# Autodesk Inventor assembly: Ensamblaje_eslabón
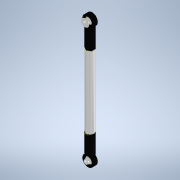
[picture p0: Inventor's stored thumbnail of the model, 180x180]
Saved by Autodesk Inventor 2020 (Build 240168000, 168)
## iProperties
Created: 2019-10-01
Part Number: Ensamblaje_eslabón
Document SubType Name: Assembly
Designer: Frederich Schnëider
Author: Frederich Schnëider
## Documents named in this file (5)
- C:\Users\Frederich Schnëider\Documents\Inventor\Eslabón TRA\Ensamblaje_eslabón.iam
- C:\Users\Frederich Schnëider\Documents\Inventor\Eslabón TRA\RCT-T003.ipt
- C:\Users\Frederich Schnëider\Documents\Inventor\Eslabón TRA\H016.ipt
- C:\Users\Frederich Schnëider\Documents\Inventor\Eslabón TRA\H016 (2).ipt
- C:\Users\Frederich Schnëider\Documents\Inventor\Eslabón TRA\RCT-T003 (2).ipt
## Components (5 placed, 4 different names)
1. RCT-T003:1 — De rotación:1, De rotación:2
2. RCT-T003 (2):1 — De rotación:2, De bola:1
3. RCT-T003 (2):2 — De rotación:1, De bola:2
4. H016:1 — De bola:2
5. H016 (2):1 — De bola:1
## Relationships (4: RevoluteJoint 2, BallJoint 2)
- De rotación:1 [RevoluteJoint]: RCT-T003:1 ↔ RCT-T003 (2):2
- De rotación:2 [RevoluteJoint]: RCT-T003:1 ↔ RCT-T003 (2):1
- De bola:2 [BallJoint]: RCT-T003 (2):2 ↔ H016:1
- De bola:1 [BallJoint]: RCT-T003 (2):1 ↔ H016 (2):1
